# Autodesk Inventor assembly: Arm for Gen 2
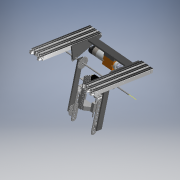
[picture p0: Inventor's stored thumbnail of the model, 180x180]
Saved by Autodesk Inventor 2019 (Build 230136000, 136)
## iProperties
Part Number: Arm for Gen 2
Document SubType Name: Assembly
Designer: Delta
Author: Delta
## Documents named in this file (11)
- C:\Robotics\CAD\2019-20_CAD\Collection\Arm for Gen 2.iam
- C:\Robotics\CAD\2019-20_CAD\Collection\12 Inch Hex Axle.ipt
- C:\Robotics\CAD\COTSParts\Sprockets - AndyMark\615106.ipt
- C:\Robotics\CAD\2019-20_CAD\Collection\bar arms.ipt
- C:\Robotics\CAD\2019-20_CAD\Collection\Spacer .25D .375H.ipt
- C:\Robotics\CAD\2019-20_CAD\Collection\Wing Left.iam
- C:\Robotics\CAD\2019-20_CAD\Collection\Wing Right.iam
- C:\Robotics\CAD\2019-20_CAD\Collection\Motor mount bar.ipt
- C:\Robotics\CAD\COTSParts\Motors\am-3643 NeveRest Sport, 104-1 with Motor.ipt
- C:\Robotics\CAD\2019-20_CAD\Collection\Motor spacer.ipt
- C:\Robotics\CAD\2019-20_CAD\Collection\The Claw.iam
## Components (13 placed, 10 different names)
1. 12 Inch Hex Axle:1 — Mate:5, Mate:6, Mate:8, Mate:55, Mate:74, Mate:80, Mate:81, Flush:10
2. 615106:1 — Mate:5, Flush:12
3. bar arms:1 — Mate:6, Flush:5, Mate:84, Mate:85, Mate:90
4. bar arms:2 — Mate:8, Flush:5, Mate:54, Mate:86, Mate:87
5. Spacer .25D .375H:1 — Mate:54, Mate:55
6. Wing Left:1 [sub-assembly] — Mate:81, Flush:10, Mate:91, Mate:92, Flush:13
7. Wing Right:1 [sub-assembly] — Mate:80, Mate:87, Mate:88, Flush:11, Mate:89, Flush:13
8. Motor mount bar:1 — Flush:8, Mate:70, Mate:79, Mate:88, Flush:11, Mate:89, Mate:91, Mate:92
9. am-3643 NeveRest Sport, 104-1 with Motor:1 — Flush:6, Flush:7, Mate:72, Mate:73, Mate:82
10. Motor spacer:1 — Flush:6, Flush:7, Flush:8, Mate:70, Mate:73, Mate:79, Angle:2
11. 615106:3 — Mate:72, Mate:82, Flush:12
12. 615106:4 — Mate:74, Mate:90
13. The Claw:1 [sub-assembly] — Mate:84, Mate:85, Mate:86, Angle:2
## Relationships (31: Mate 22, Flush 8, Angle 1)
- Mate:5: 12 Inch Hex Axle:1 ↔ 615106:1
- Mate:6: 12 Inch Hex Axle:1 ↔ bar arms:1
- Mate:8: 12 Inch Hex Axle:1 ↔ bar arms:2
- Flush:5: bar arms:1 ↔ bar arms:2
- Mate:54: bar arms:2 ↔ Spacer .25D .375H:1
- Mate:55: 12 Inch Hex Axle:1 ↔ Spacer .25D .375H:1
- Flush:6: am-3643 NeveRest Sport, 104-1 with Motor:1 ↔ Motor spacer:1
- Flush:7: am-3643 NeveRest Sport, 104-1 with Motor:1 ↔ Motor spacer:1
- Flush:8: Motor mount bar:1 ↔ Motor spacer:1
- Mate:70: Motor mount bar:1 ↔ Motor spacer:1
- Mate:72: am-3643 NeveRest Sport, 104-1 with Motor:1 ↔ 615106:3
- Mate:73: am-3643 NeveRest Sport, 104-1 with Motor:1 ↔ Motor spacer:1
- Mate:74: 12 Inch Hex Axle:1 ↔ 615106:4
- Mate:79: Motor mount bar:1 ↔ Motor spacer:1
- Mate:80: 12 Inch Hex Axle:1 ↔ Wing Right:1
- Mate:81: 12 Inch Hex Axle:1 ↔ Wing Left:1
- Mate:82 (25.4 mm): am-3643 NeveRest Sport, 104-1 with Motor:1 ↔ 615106:3
- Flush:10 (-71.628 mm): 12 Inch Hex Axle:1 ↔ Wing Left:1
- Mate:84: bar arms:1 ↔ The Claw:1
- Mate:85: bar arms:1 ↔ The Claw:1
- Mate:86: bar arms:2 ↔ The Claw:1
- Angle:2 (0 deg): Motor spacer:1 ↔ The Claw:1
- Mate:87 (19.5326 mm): bar arms:2 ↔ Wing Right:1
- Mate:88: Wing Right:1 ↔ Motor mount bar:1
- Flush:11: Wing Right:1 ↔ Motor mount bar:1
- Mate:89: Wing Right:1 ↔ Motor mount bar:1
- Mate:90 (9.6266 mm): bar arms:1 ↔ 615106:4
- Flush:12: 615106:1 ↔ 615106:3
- Mate:91: Wing Left:1 ↔ Motor mount bar:1
- Mate:92: Wing Left:1 ↔ Motor mount bar:1
- Flush:13: Wing Left:1 ↔ Wing Right:1
